# Autodesk Inventor assembly: Shaft Collar Metal
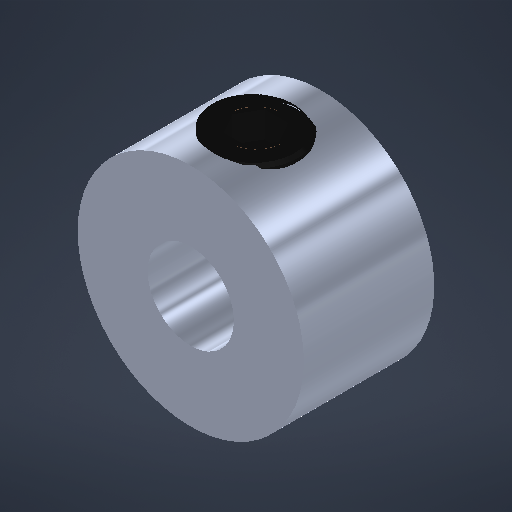
[picture p0: Inventor's stored thumbnail of the model, 512x512]
Saved by Autodesk Inventor 2025.2 (Build 292293000, 293)
## iProperties
Created: 2022-08-01
Part Number: Shaft Collar Metal
Document SubType Name: Assembly
Designer: ylu12
Author: ylu12
## Documents named in this file (4)
- C:\1629X-7700R-Worlds-Bot\VEX-CAD-Inventor-1.4.2\Motion\Shaft LS\Shaft Collar Metal\Shaft Collar Set Screw.iam
- C:\1629X-7700R-Worlds-Bot\VEX-CAD-Inventor-1.4.2\Motion\Reference Files\Shaft Collar Metal.ipt
- C:\1629X-7700R-Worlds-Bot\VEX-CAD-Inventor-1.4.2\Motion\Reference Files\Set Screw.ipt
- C:\1629X-7700R-Worlds-Bot\VEX-CAD-Inventor-1.4.2\Motion\Shaft LS\Shaft Collar Metal.iam
## Components (2 placed, 2 different names)
1. Shaft Collar Metal:1 — Mate:1, Mate:2, Flush:1, Insert:1
2. Set Screw:1 — Insert:1
## Relationships (4: Mate 2, Flush 1, Insert 1)
- Mate:1: Shaft Collar Metal:1
- Mate:2: Shaft Collar Metal:1
- Flush:1: Shaft Collar Metal:1
- Insert:1: Shaft Collar Metal:1 ↔ Set Screw:1
